# Autodesk Inventor assembly: Assembly of Parts
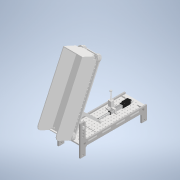
[picture p0: Inventor's stored thumbnail of the model, 180x180]
Saved by Autodesk Inventor 2022 (Build 260153000, 153)
## iProperties
Created: 2022-01-26
Part Number: Assembly of Parts
Document SubType Name: Assembly
Designer: owner
Author: owner
## Documents named in this file (18)
- D:\McMaster University\Engineering 1\Year 1\Winter 2022 Term\ENGINEER 1P13B\Projects\Project 3\Final Design\Thurs-39_P3_CAD_Files\Assembly of Parts.iam
- D:\McMaster University\Engineering 1\Year 1\Winter 2022 Term\ENGINEER 1P13B\Projects\Project 3\Final Design\Thurs-39_P3_CAD_Files\Baseplate - Metric Holes.iam
- D:\McMaster University\Engineering 1\Year 1\Winter 2022 Term\ENGINEER 1P13B\Projects\Project 3\Final Design\Thurs-39_P3_CAD_Files\Hopper_And_Connecting_Plate.iam
- D:\McMaster University\Engineering 1\Year 1\Winter 2022 Term\ENGINEER 1P13B\Projects\Project 3\Final Design\Thurs-39_P3_CAD_Files\0.25 Inch x 4.5 inch Bolt.ipt
- D:\McMaster University\Engineering 1\Year 1\Winter 2022 Term\ENGINEER 1P13B\Projects\Project 3\Final Design\Thurs-39_P3_CAD_Files\0.25 Inch Nut.ipt
- D:\McMaster University\Engineering 1\Year 1\Winter 2022 Term\ENGINEER 1P13B\Projects\Project 3\Final Design\Thurs-39_P3_CAD_Files\Linear Actuator.iam
- D:\McMaster University\Engineering 1\Year 1\Winter 2022 Term\ENGINEER 1P13B\Projects\Project 3\Final Design\Thurs-39_P3_CAD_Files\Linear Actuator Rear Mount.ipt
- D:\McMaster University\Engineering 1\Year 1\Winter 2022 Term\ENGINEER 1P13B\Projects\Project 3\Final Design\Thurs-39_P3_CAD_Files\M4 x 16mm Machine Screw.ipt
- D:\McMaster University\Engineering 1\Year 1\Winter 2022 Term\ENGINEER 1P13B\Projects\Project 3\Final Design\Thurs-39_P3_CAD_Files\Linear Actuator Mount.ipt
- D:\McMaster University\Engineering 1\Year 1\Winter 2022 Term\ENGINEER 1P13B\Projects\Project 3\Final Design\Thurs-39_P3_CAD_Files\M4 Nut.ipt
- D:\McMaster University\Engineering 1\Year 1\Winter 2022 Term\ENGINEER 1P13B\Projects\Project 3\Final Design\Thurs-39_P3_CAD_Files\Hopper Rest 8-32.iam
- D:\McMaster University\Engineering 1\Year 1\Winter 2022 Term\ENGINEER 1P13B\Projects\Project 3\Final Design\Thurs-39_P3_CAD_Files\Rod.ipt
- D:\McMaster University\Engineering 1\Year 1\Winter 2022 Term\ENGINEER 1P13B\Projects\Project 3\Final Design\Thurs-39_P3_CAD_Files\Cylindrical Pin Actuator Piece.ipt
- D:\McMaster University\Engineering 1\Year 1\Winter 2022 Term\ENGINEER 1P13B\Projects\Project 3\Final Design\Thurs-39_P3_CAD_Files\M4 x 20mm Machine Screw.ipt
- D:\McMaster University\Engineering 1\Year 1\Winter 2022 Term\ENGINEER 1P13B\Projects\Project 3\Final Design\Thurs-39_P3_CAD_Files\Pin Securing Piece.ipt
- D:\McMaster University\Engineering 1\Year 1\Winter 2022 Term\ENGINEER 1P13B\Projects\Project 3\Final Design\Thurs-39_P3_CAD_Files\92095A198_Button Head Hex Drive Screw.ipt
- D:\McMaster University\Engineering 1\Year 1\Winter 2022 Term\ENGINEER 1P13B\Projects\Project 3\Final Design\Thurs-39_P3_CAD_Files\Slider7.ipt
- D:\McMaster University\Engineering 1\Year 1\Winter 2022 Term\ENGINEER 1P13B\Projects\Project 3\Final Design\Thurs-39_P3_CAD_Files\Cylindrical Pin.ipt
## Components (37 placed, 17 different names)
1. Baseplate - Metric Holes:1 [sub-assembly] — Insert:1, Mate:2, Angle:1, Mate:3, Mate:4, Mate:5, Mate:6, Mate:7, Mate:9, Mate:10, Mate:11, Mate:12, Mate:13, Mate:14
2. Hopper_And_Connecting_Plate:1 [sub-assembly] — Mate:1, Mate:2, Angle:1, Insert:23, Insert:26
3. 0.25 Inch x 4.5 inch Bolt:1 — Insert:1, Mate:1, Insert:2
4. 0.25 Inch Nut:1 — Insert:2
5. Linear Actuator:1 [sub-assembly] — Mate:3, Mate:4, Mate:8, Mate:15, Mate:16
6. Linear Actuator Rear Mount:1 — Mate:5, Mate:6, Mate:7, Insert:3, Mate:8, Insert:4
7. M4 x 16mm Machine Screw:1 — Insert:4, Insert:7
8. M4 x 16mm Machine Screw:2 — Insert:3, Insert:8
9. M4 x 16mm Machine Screw:3 — Insert:6, Insert:10
10. M4 x 16mm Machine Screw:4 — Insert:5, Insert:9
11. Linear Actuator Mount:1 — Mate:9, Mate:10, Mate:11, Insert:5, Insert:6
12. M4 Nut:1 — Insert:10
13. M4 Nut:2 — Insert:9
14. M4 Nut:3 — Insert:8
15. M4 Nut:4 — Insert:7
16. Hopper Rest 8-32:1 [sub-assembly] — Mate:12, Mate:13, Mate:14, Insert:12, Insert:13
17. Rod:1 — Insert:16, Mate:16, Insert:27
18. Cylindrical Pin Actuator Piece:1 — Insert:16, Mate:15, Insert:17, Insert:18
19. M4 Nut:5 — Insert:15
20. M4 Nut:6 — Insert:14
21. M4 x 20mm Machine Screw:1 — Insert:13, Insert:15
22. M4 x 20mm Machine Screw:2 — Insert:12, Insert:14
23. Pin Securing Piece:1 — Insert:18
24. Pin Securing Piece:2 — Insert:17
25. 92095A198_Button Head Hex Drive Screw:1 — Insert:24, Insert:26, Insert:31
26. 92095A198_Button Head Hex Drive Screw:2 — Insert:25, Insert:30
27. 92095A198_Button Head Hex Drive Screw:3 — Insert:21, Insert:28
28. 92095A198_Button Head Hex Drive Screw:4 — Insert:22, Insert:23, Insert:29
29. Cylindrical Pin:1 — Insert:27, Mate:17, Insert:32, Insert:33
30. M4 Nut:7 — Insert:30
31. M4 Nut:8 — Insert:29
32. M4 Nut:9 — Insert:31
33. M4 Nut:10 — Insert:28
34. Pin Securing Piece:3 — Insert:32
35. Pin Securing Piece:4 — Insert:33
36. Slider7:1 — Insert:21, Insert:22
37. Slider7:2 — Insert:24, Insert:25, Mate:17
## Relationships (48: Insert 30, Mate 17, Angle 1)
- Insert:1: Baseplate - Metric Holes:1 ↔ 0.25 Inch x 4.5 inch Bolt:1
- Mate:1: Hopper_And_Connecting_Plate:1 ↔ 0.25 Inch x 4.5 inch Bolt:1
- Mate:2 (2.715 mm): Baseplate - Metric Holes:1 ↔ Hopper_And_Connecting_Plate:1
- Angle:1 (0 deg): Baseplate - Metric Holes:1 ↔ Hopper_And_Connecting_Plate:1
- Insert:2 (4.0338 mm): 0.25 Inch x 4.5 inch Bolt:1 ↔ 0.25 Inch Nut:1
- Mate:3: Baseplate - Metric Holes:1 ↔ Linear Actuator:1
- Mate:4 (38.855 mm): Baseplate - Metric Holes:1 ↔ Linear Actuator:1
- Mate:5: Baseplate - Metric Holes:1 ↔ Linear Actuator Rear Mount:1
- Mate:6 (40.705 mm): Baseplate - Metric Holes:1 ↔ Linear Actuator Rear Mount:1
- Mate:7: Baseplate - Metric Holes:1 ↔ Linear Actuator Rear Mount:1
- Insert:3: Linear Actuator Rear Mount:1 ↔ M4 x 16mm Machine Screw:2
- Mate:8: Linear Actuator:1 ↔ Linear Actuator Rear Mount:1
- Insert:4 (4.7 mm): Linear Actuator Rear Mount:1 ↔ M4 x 16mm Machine Screw:1
- Mate:9: Baseplate - Metric Holes:1 ↔ Linear Actuator Mount:1
- Mate:10: Baseplate - Metric Holes:1 ↔ Linear Actuator Mount:1
- Mate:11: Baseplate - Metric Holes:1 ↔ Linear Actuator Mount:1
- Insert:5: M4 x 16mm Machine Screw:4 ↔ Linear Actuator Mount:1
- Insert:6: M4 x 16mm Machine Screw:3 ↔ Linear Actuator Mount:1
- Insert:7 (1 mm): M4 x 16mm Machine Screw:1 ↔ M4 Nut:4
- Insert:8 (5.7 mm): M4 x 16mm Machine Screw:2 ↔ M4 Nut:3
- Insert:9 (-6.2 mm): M4 x 16mm Machine Screw:4 ↔ M4 Nut:2
- Insert:10 (-6.2 mm): M4 x 16mm Machine Screw:3 ↔ M4 Nut:1
- Mate:12: Baseplate - Metric Holes:1 ↔ Hopper Rest 8-32:1
- Mate:13: Baseplate - Metric Holes:1 ↔ Hopper Rest 8-32:1
- Mate:14: Baseplate - Metric Holes:1 ↔ Hopper Rest 8-32:1
- Insert:12: Hopper Rest 8-32:1 ↔ M4 x 20mm Machine Screw:2
- Insert:13: Hopper Rest 8-32:1 ↔ M4 x 20mm Machine Screw:1
- Insert:14 (3.9 mm): M4 Nut:6 ↔ M4 x 20mm Machine Screw:2
- Insert:15 (3.9 mm): M4 Nut:5 ↔ M4 x 20mm Machine Screw:1
- Insert:16 (-31 mm): Rod:1 ↔ Cylindrical Pin Actuator Piece:1
- Mate:15: Linear Actuator:1 ↔ Cylindrical Pin Actuator Piece:1
- Mate:16 (4 mm): Linear Actuator:1 ↔ Rod:1
- Insert:17 (-9 mm): Cylindrical Pin Actuator Piece:1 ↔ Pin Securing Piece:2
- Insert:18 (-9 mm): Cylindrical Pin Actuator Piece:1 ↔ Pin Securing Piece:1
- Insert:21: 92095A198_Button Head Hex Drive Screw:3 ↔ Slider7:1
- Insert:22: 92095A198_Button Head Hex Drive Screw:4 ↔ Slider7:1
- Insert:23 (12.7 mm): Hopper_And_Connecting_Plate:1 ↔ 92095A198_Button Head Hex Drive Screw:4
- Insert:24: 92095A198_Button Head Hex Drive Screw:1 ↔ Slider7:2
- Insert:25: 92095A198_Button Head Hex Drive Screw:2 ↔ Slider7:2
- Insert:26 (12.7 mm): Hopper_And_Connecting_Plate:1 ↔ 92095A198_Button Head Hex Drive Screw:1
- Insert:27 (-42.625 mm): Rod:1 ↔ Cylindrical Pin:1
- Insert:28 (7.5 mm): 92095A198_Button Head Hex Drive Screw:3 ↔ M4 Nut:10
- Insert:29 (8 mm): 92095A198_Button Head Hex Drive Screw:4 ↔ M4 Nut:8
- Insert:30 (7.5 mm): 92095A198_Button Head Hex Drive Screw:2 ↔ M4 Nut:7
- Insert:31 (7.6 mm): 92095A198_Button Head Hex Drive Screw:1 ↔ M4 Nut:9
- Mate:17: Cylindrical Pin:1 ↔ Slider7:2
- Insert:32 (-10.225 mm): Cylindrical Pin:1 ↔ Pin Securing Piece:3
- Insert:33 (-10.225 mm): Cylindrical Pin:1 ↔ Pin Securing Piece:4
